# Autodesk Inventor assembly: bearing block wheel mount inner
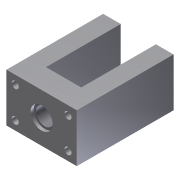
[picture p0: Inventor's stored thumbnail of the model, 180x180]
Saved by Autodesk Inventor 2012 (Build 160160000, 160)
## iProperties
Created: 2012-04-26
Part Number: bearing block wheel mount inner
Document SubType Name: Assembly
Designer: Antonella Wilby
Author: Antonella Wilby
## Documents named in this file (4)
- C:\Users\Antonella\Documents\GCC Robotics 2012 - Mechanical\Robot 2.0\Drive Train\bearing block wheel mount inner.iam
- C:\Users\Antonella\Documents\GCC Robotics 2012 - Mechanical\Robot 2.0\Drive Train\mount pillow block inner.ipt
- C:\Users\Antonella\Documents\GCC Robotics 2012 - Mechanical\Robot 2.0\Drive Train\R8-ZZ.ipt
- C:\Users\Antonella\Documents\GCC Robotics 2012 - Mechanical\Robot 2.0\Drive Train\mount pillow block inner bearing capture.ipt
## Components (3 placed, 3 different names)
1. mount pillow block inner:1 — Mate:1, Mate:2, Mate:3, Mate:5
2. R8-ZZ:1 — Mate:1, Mate:2, Mate:4
3. mount pillow block inner bearing capture:1 — Mate:3, Mate:4, Mate:5
## Relationships (5: Mate 5)
- Mate:1: mount pillow block inner:1 ↔ R8-ZZ:1
- Mate:2: mount pillow block inner:1 ↔ R8-ZZ:1
- Mate:3: mount pillow block inner:1 ↔ mount pillow block inner bearing capture:1
- Mate:4: R8-ZZ:1 ↔ mount pillow block inner bearing capture:1
- Mate:5: mount pillow block inner:1 ↔ mount pillow block inner bearing capture:1
